# Autodesk Inventor assembly: AMT103Encoder
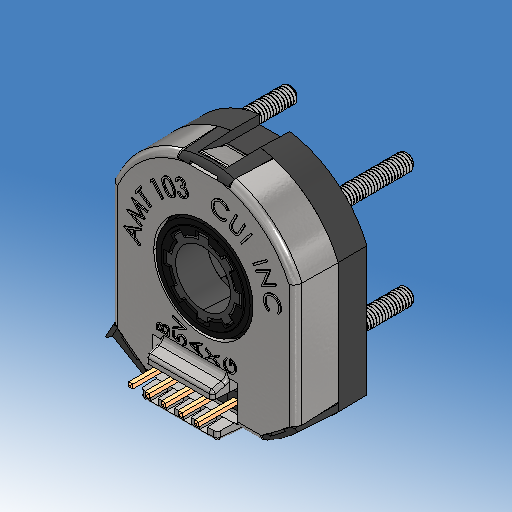
[picture p0: Inventor's stored thumbnail of the model, 512x512]
Saved by Autodesk Inventor 2025 (Build 290162000, 162)
## iProperties
Created: 2024-06-19
Part Number: AMT103Encoder
Document SubType Name: Assembly
Designer: seene
Author: seene
## Documents named in this file (4)
- C:\Users\seene\Desktop\Stony Brook\SBRT\RCR_Dexter\Drive\v1\AMT103Encoder.iam
- C:\Users\seene\Desktop\Stony Brook\SBRT\RCR_Dexter\Drive\v1\amt103-v_25 MODIFIED FOR TETRIX(2).ipt
- C:\Users\seene\Desktop\Stony Brook\SBRT\RCR_Dexter\Drive\v1\amt103-v unit only.ipt
- C:\Users\seene\Desktop\Stony Brook\SBRT\RCR_Dexter\Drive\v1\93395A185_316 Stainless Steel Hex Drive Flat Head Screw.ipt
## Components (6 placed, 3 different names)
1. amt103-v_25 MODIFIED FOR TETRIX(2):1 — Mate:1, Mate:2, Mate:3, Flush:1
2. amt103-v unit only:1 — Mate:1, Mate:2
3. 93395A185_316 Stainless Steel Hex Drive Flat Head Screw:1 — Mate:3, Flush:1
4. 93395A185_316 Stainless Steel Hex Drive Flat Head Screw:2
5. 93395A185_316 Stainless Steel Hex Drive Flat Head Screw:3
6. 93395A185_316 Stainless Steel Hex Drive Flat Head Screw:4
## Component patterns: (4 elements, first: 93395A185_316 Stainless Steel Hex Drive Flat Head Screw:1)
## Relationships (4: Mate 3, Flush 1)
- Mate:1: amt103-v_25 MODIFIED FOR TETRIX(2):1 ↔ amt103-v unit only:1
- Mate:2: amt103-v_25 MODIFIED FOR TETRIX(2):1 ↔ amt103-v unit only:1
- Mate:3: amt103-v_25 MODIFIED FOR TETRIX(2):1 ↔ 93395A185_316 Stainless Steel Hex Drive Flat Head Screw:1
- Flush:1: amt103-v_25 MODIFIED FOR TETRIX(2):1 ↔ 93395A185_316 Stainless Steel Hex Drive Flat Head Screw:1
